# Autodesk Inventor assembly: ASY Beshkino_bio_tank
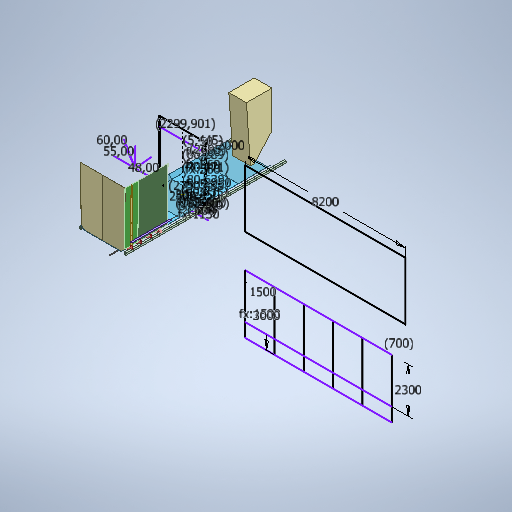
[picture p0: Inventor's stored thumbnail of the model, 512x512]
Saved by Autodesk Inventor 2025 (Build 290162010, 162A)
## iProperties
Created: 2024-07-21
Part Number: ASY Beshkino_bio_tank
Document SubType Name: Assembly
Designer: admin
Author: admin
## Documents named in this file (12)
- C:\Users\admin\YandexDisk-badmisterfox\домашниий пк\Inventor\BSH_Beshkino_bio_tank\ASY Beshkino_bio_tank.iam
- C:\Users\admin\YandexDisk-badmisterfox\домашниий пк\Inventor\BSH_Beshkino_bio_tank\BSH 000 dim Beshkino_bio_tank.ipt
- C:\Users\admin\YandexDisk-badmisterfox\домашниий пк\Inventor\BSH_Beshkino_bio_tank\BSH 010 floor 1.ipt
- C:\Users\admin\YandexDisk-badmisterfox\домашниий пк\Inventor\BSH_Beshkino_bio_tank\BSH 021 rib 1.ipt
- C:\Users\admin\YandexDisk-badmisterfox\домашниий пк\Inventor\BSH_Beshkino_bio_tank\BSH 022 rib 2.ipt
- C:\Users\admin\YandexDisk-badmisterfox\домашниий пк\Inventor\BSH_Beshkino_bio_tank\BSH 061 tube 1.ipt
- C:\Users\admin\YandexDisk-badmisterfox\домашниий пк\Inventor\BSH_Beshkino_bio_tank\BSH 031 nose 1.ipt
- C:\Users\admin\YandexDisk-badmisterfox\домашниий пк\Inventor\BSH_Beshkino_bio_tank\BSH 032 board 2.ipt
- C:\Users\admin\YandexDisk-badmisterfox\домашниий пк\Inventor\BSH_Beshkino_bio_tank\BSH 033 board 3.ipt
- C:\Users\admin\YandexDisk-badmisterfox\домашниий пк\Inventor\BSH_Beshkino_bio_tank\BSH 041 stringer 1.ipt
- C:\Users\admin\YandexDisk-badmisterfox\домашниий пк\Inventor\BSH_Beshkino_bio_tank\BSH 039 back 9.ipt
- C:\Users\admin\YandexDisk-badmisterfox\домашниий пк\Inventor\BSH_Beshkino_bio_tank\BSH 041 stringer floor.ipt
## Components (21 placed, 11 different names)
1. BSH 000 dim Beshkino_bio_tank:1
2. BSH 010 floor 1:1 — Mate:5, Mate:6, Rigid:4, Mate:7, Flush:4, Mate:10, Flush:5
3. BSH 020 rib 1:1 — Mate:4, Flush:3, Mate:5, Mate:6, Rigid:3, Rigid:9
4. BSH 022 rib 2:1 — Rigid:3, Mate:8
5. BSH 061 tube 1:1 — Mate:1, Rigid:1, Mate:3, Flush:6
6. BSH 061 tube 1:2 — Mate:2, Rigid:1, Mate:4, Flush:3, Flush:4, Flush:14, Mate:14
7. BSH 031 nose 1:1 — Mate:10, Flush:5, Mate:11, Rigid:11
8. BSH 010 floor 1:2 — Rigid:4, Rigid:5
9. BSH 010 floor 1:3 — Rigid:5, Rigid:6, Mate:9
10. BSH 010 floor 1:4 — Rigid:6, Rigid:7
11. BSH 010 floor 1:5 — Rigid:7, Mate:12
12. BSH 032 board 2:1 — Mate:8, Mate:9, Rigid:8
13. BSH 033 board 3:1 — Rigid:8
14. BSH 020 rib 1:3 — Rigid:9, Rigid:10
15. BSH 020 rib 1:4 — Rigid:10, Rigid:12
16. BSH 031 nose 1:2 — Rigid:11
17. BSH 041 stringer 1:1
18. BSH 039 back 9:1 — Mate:12, Flush:6
19. BSH 020 rib 1:5 — Flush:14, Mate:14, Rigid:13
20. BSH 041 stringer floor:1 — Rigid:12
21. BSH 041 stringer floor:2 — Rigid:13
## Relationships (30: Mate 13, WeldJoint 12, Flush 5)
- Mate:1: BSH 061 tube 1:1
- Mate:2: BSH 061 tube 1:2
- Rigid:1 [WeldJoint] (-2400 mm): BSH 061 tube 1:1 ↔ BSH 061 tube 1:2
- Mate:3: BSH 061 tube 1:1
- Mate:4: BSH 020 rib 1:1 ↔ BSH 061 tube 1:2
- Flush:3: BSH 020 rib 1:1 ↔ BSH 061 tube 1:2
- Mate:5: BSH 010 floor 1:1 ↔ BSH 020 rib 1:1
- Mate:6: BSH 010 floor 1:1 ↔ BSH 020 rib 1:1
- Rigid:3 [WeldJoint]: BSH 020 rib 1:1 ↔ BSH 022 rib 2:1
- Rigid:4 [WeldJoint]: BSH 010 floor 1:1 ↔ BSH 010 floor 1:2
- Rigid:5 [WeldJoint]: BSH 010 floor 1:2 ↔ BSH 010 floor 1:3
- Rigid:6 [WeldJoint]: BSH 010 floor 1:3 ↔ BSH 010 floor 1:4
- Rigid:7 [WeldJoint]: BSH 010 floor 1:4 ↔ BSH 010 floor 1:5
- Mate:7: BSH 010 floor 1:1
- Flush:4: BSH 010 floor 1:1 ↔ BSH 061 tube 1:2
- Mate:8: BSH 022 rib 2:1 ↔ BSH 032 board 2:1
- Mate:9: BSH 010 floor 1:3 ↔ BSH 032 board 2:1
- Rigid:8 [WeldJoint]: BSH 032 board 2:1 ↔ BSH 033 board 3:1
- Rigid:9 [WeldJoint] (-500 mm): BSH 020 rib 1:1 ↔ BSH 020 rib 1:3
- Rigid:10 [WeldJoint] (-500 mm): BSH 020 rib 1:3 ↔ BSH 020 rib 1:4
- Mate:10: BSH 010 floor 1:1 ↔ BSH 031 nose 1:1
- Flush:5 (10 mm): BSH 010 floor 1:1 ↔ BSH 031 nose 1:1
- Mate:11: BSH 031 nose 1:1
- Rigid:11 [WeldJoint]: BSH 031 nose 1:1 ↔ BSH 031 nose 1:2
- Mate:12: BSH 010 floor 1:5 ↔ BSH 039 back 9:1
- Flush:6: BSH 061 tube 1:1 ↔ BSH 039 back 9:1
- Flush:14: BSH 061 tube 1:2 ↔ BSH 020 rib 1:5
- Mate:14: BSH 061 tube 1:2 ↔ BSH 020 rib 1:5
- Rigid:12 [WeldJoint]: BSH 020 rib 1:4 ↔ BSH 041 stringer floor:1
- Rigid:13 [WeldJoint]: BSH 020 rib 1:5 ↔ BSH 041 stringer floor:2
